# Autodesk Inventor assembly: Chassis-ver11-1111-2019
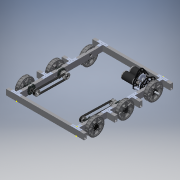
[picture p0: Inventor's stored thumbnail of the model, 180x180]
Saved by Autodesk Inventor 2018 (Build 220112000, 112)
## iProperties
Created: 2019-10-10
Part Number: Chassis-ver11-1111-2019
Document SubType Name: Assembly
Designer: JMHal
Author: JMHal
## Documents named in this file (26)
- E:\GrabCad\2020 Infinite Recharge\Chassis\Assembly\Chassis-ver11-1111-2019.iam
- E:\GrabCad\2020 Infinite Recharge\Chassis\Parts\2x1 20in Alluminum with Cal Drop.ver1-1111-2019.ipt
- E:\GrabCad\2020 Infinite Recharge\Chassis\Parts\2x1 20in Alluminum.ver1-1111-2019.ipt
- E:\GrabCad\2020 Infinite Recharge\Chassis\Parts\2x1 2in Alluminum Block.ver1-1111-2019.ipt
- E:\GrabCad\Resources\VEXpro Resources\Bearings\0.5inHexFlangedBearing(1.125inx0.313in)-1111-2016.ipt
- E:\GrabCad\Resources\VEXpro Resources\Versa Motion\VersaBlockKit-1111-2016.ipt
- E:\GrabCad\Resources\VEXpro Resources\Shafts\0.5inThunderHexShaft(8)-1111-2016.ipt
- E:\GrabCad\Resources\VEXpro Resources\Gearboxes\WCP SS Gearbox\SS-Gearbox.iam
- E:\GrabCad\Resources\VEXpro Resources\Gussets\ChassisGusset-1111-2016.ipt
- E:\GrabCad\2020 Infinite Recharge\Chassis\Parts\ElectricalBoard.ver1-1111-2019.ipt
- E:\GrabCad\Resources\VEXpro Resources\Spacers\0.5inAcetalSpace(0.5inHex)-1111-2016.ipt
- E:\GrabCad\Resources\VEXpro Resources\Spacers\0.5inAcetalSpace(0.5inHex)-1111-2016_MIR.ipt
- E:\GrabCad\Resources\VEXpro Resources\Versa Motion\Timing Pulleys\TimingPulley30T15mmDoubleFlange(0.5inHex)-1111-2017.ipt
- E:\GrabCad\Resources\VEXpro Resources\Spacers\0.25inAcetalSpacer(0.5inHex)-1111-2016.ipt
- E:\GrabCad\Resources\VEXpro Resources\Spacers\0.125inAcetalSpacer(0.5inHex)-1111-2016.ipt
- E:\GrabCad\Resources\VEXpro Resources\Spacers\0.0625inAcetalSpacer(0.5inHex)-1111-2016.ipt
- E:\GrabCad\Resources\VEXpro Resources\Spacers\1inAcetalSpacer(0.5inHex)-1111-2016.ipt
- E:\GrabCad\Resources\VEXpro Resources\Versa Motion\Timing Pulleys\TimingPulley30T15mmDoubleFlange(0.5inHex)-1111-2017_MIR.ipt
- E:\GrabCad\Resources\VEXpro Resources\Spacers\0.25inAcetalSpacer(0.5inHex)-1111-2016_MIR.ipt
- E:\GrabCad\Resources\VEXpro Resources\Spacers\0.125inAcetalSpacer(0.5inHex)-1111-2016_MIR.ipt
- E:\GrabCad\Resources\VEXpro Resources\Spacers\0.0625inAcetalSpacer(0.5inHex)-1111-2016_MIR.ipt
- E:\GrabCad\Resources\VEXpro Resources\Spacers\1inAcetalSpacer(0.5inHex)-1111-2016_MIR.ipt
- E:\GrabCad\2020 Infinite Recharge\Chassis\Parts\BeltVer1-1111-2019.ipt
- E:\GrabCad\Resources\VEXpro Resources\Wheels\6 inch\6x1inTractionWheel-1111-2016.iam
- E:\GrabCad\2020 Infinite Recharge\Chassis\Parts\Bumbers.ver1-1111-2019.ipt
- C:\Users\Demarcus\Desktop\WCDShiftingGearboxPTO.ver1-1111-2020.iam
## Components (69 placed, 25 different names)
1. 2x1 20in Alluminum with Cal Drop.ver1-1111-2019:1 — Mate:31, Mate:32, Insert:7, Mate:51, Insert:8, Angle:2, Mate:53, Angle:9, Insert:17, Angle:10, Insert:19, Angle:11, Mate:60, Cylindrical:1, Angle:16, Flush:1, Mate:65, Mate:66, Flush:2, Mate:67, Flush:4, Flush:5, Mate:77, Mate:78, Flush:16, Flush:17, Mate:80, Flush:20, Flush:23, Symmetry:1, Flush:43, Symmetry:2, Flush:62, Mate:141
2. 2x1 20in Alluminum.ver1-1111-2019:1 — Mate:65, Mate:66, Flush:2, Mate:68, Mate:72, Mate:81, Flush:22, Mate:82, Flush:24, Flush:44, Flush:62, Mate:140, Flush:63
3. 2x1 20in Alluminum with Cal Drop.ver1-1111-2019:2 — Insert:4, Insert:5, Angle:7, Angle:8, Insert:23, Angle:13, Insert:25, Angle:14, Flush:6, Flush:8, Mate:73, Flush:9, Flush:34, Flush:35, Flush:36, Flush:37, Symmetry:1, Symmetry:2, Cylindrical:42, Mate:142, Mate:143
4. 2x1 20in Alluminum.ver1-1111-2019:2 — Mate:67, Flush:4, Flush:5, Mate:69, Flush:6, Mate:71, Mate:73, Mate:79, Flush:19, Flush:21
5. 0.5inThunderHexShaft(8)-1111-2016:1 — Cylindrical:2, Cylindrical:18
6. SS-Gearbox:2 [sub-assembly] — Mate:60, Cylindrical:1, Angle:16
7. 0.5inThunderHexShaft(8)-1111-2016:2 — Cylindrical:3, Cylindrical:16, Flush:64
8. ChassisGusset-1111-2016:1 — Mate:76, Flush:12, Flush:36
9. ChassisGusset-1111-2016:2 — Mate:75, Flush:11, Flush:35
10. ChassisGusset-1111-2016:3 — Mate:78, Flush:14, Flush:17
11. ChassisGusset-1111-2016:4 — Mate:77, Flush:15, Flush:16
12. ChassisGusset-1111-2016:5 — Mate:82, Flush:24, Flush:34
13. ChassisGusset-1111-2016:6 — Mate:81, Flush:22, Flush:23
14. ChassisGusset-1111-2016:7 — Mate:80, Flush:20, Flush:21
15. ChassisGusset-1111-2016:8 — Mate:79, Flush:19, Flush:37
16. ElectricalBoard.ver1-1111-2019:1 — Flush:43, Flush:44
17. 0.5inAcetalSpace(0.5inHex)-1111-2016:1 — Cylindrical:16, Mate:89, Cylindrical:34, Mate:130
18. 0.5inAcetalSpace(0.5inHex)-1111-2016:2 — Cylindrical:18, Mate:91, Cylindrical:35, Mate:131
19. 0.25inAcetalSpacer(0.5inHex)-1111-2016:3 — Cylindrical:36, Mate:132
20. 0.5inAcetalSpace(0.5inHex)-1111-2016_MIR:1 — Mate:119, Rotational:14, Cylindrical:38, Mate:134
21. 0.5inAcetalSpace(0.5inHex)-1111-2016_MIR:2 — Cylindrical:31, Mate:127, Rotational:15
22. 0.25inAcetalSpacer(0.5inHex)-1111-2016:4 — Cylindrical:40, Mate:136
23. TimingPulley30T15mmDoubleFlange(0.5inHex)-1111-2017:1 — Rotational:7, Mate:117
24. TimingPulley30T15mmDoubleFlange(0.5inHex)-1111-2017:2 — Rotational:3
25. TimingPulley30T15mmDoubleFlange(0.5inHex)-1111-2017:3 — Cylindrical:25, Mate:111, Rotational:2
26. 0.25inAcetalSpacer(0.5inHex)-1111-2016:1 — Cylindrical:25, Cylindrical:26, Mate:109, Mate:110, Rotational:4
27. 0.125inAcetalSpacer(0.5inHex)-1111-2016:1 — Cylindrical:26, Mate:110, Mate:111
28. 0.0625inAcetalSpacer(0.5inHex)-1111-2016:1 — Rotational:2, Rotational:3
29. 0.25inAcetalSpacer(0.5inHex)-1111-2016:2 — Rotational:6, Rotational:7
30. 1inAcetalSpacer(0.5inHex)-1111-2016:1 — Rotational:5, Rotational:6
31. TimingPulley30T15mmDoubleFlange(0.5inHex)-1111-2017_MIR:1 — Rotational:10, Mate:114, Mate:115
32. TimingPulley30T15mmDoubleFlange(0.5inHex)-1111-2017_MIR:2 — Rotational:8, Cylindrical:30, Flush:60
33. TimingPulley30T15mmDoubleFlange(0.5inHex)-1111-2017_MIR:3 — Mate:112, Cylindrical:27, Rotational:9
34. 0.25inAcetalSpacer(0.5inHex)-1111-2016_MIR:1 — Mate:113, Cylindrical:27, Cylindrical:28, Rotational:12
35. 0.125inAcetalSpacer(0.5inHex)-1111-2016_MIR:1 — Mate:112, Mate:113, Cylindrical:28
36. 0.0625inAcetalSpacer(0.5inHex)-1111-2016_MIR:1 — Rotational:8, Rotational:9
37. 0.25inAcetalSpacer(0.5inHex)-1111-2016_MIR:2 — Rotational:10, Rotational:11
38. 1inAcetalSpacer(0.5inHex)-1111-2016_MIR:1 — Rotational:11, Rotational:13
39. BeltVer1-1111-2019:1 — Mate:114, Mate:115
40. BeltVer1-1111-2019:2 — Mate:117
41. 0.5inThunderHexShaft(8)-1111-2016:3 — Cylindrical:30, Flush:60, Cylindrical:31
42. 6x1inTractionWheel-1111-2016:1 [sub-assembly] — Cylindrical:34, Mate:130, Flush:64
43. 6x1inTractionWheel-1111-2016:2 [sub-assembly] — Cylindrical:35, Mate:131
44. 6x1inTractionWheel-1111-2016:3 [sub-assembly] — Cylindrical:36, Mate:132
45. 6x1inTractionWheel-1111-2016:5 [sub-assembly] — Cylindrical:38, Mate:134
46. 6x1inTractionWheel-1111-2016:6 [sub-assembly] — Cylindrical:40, Mate:136
47. 6x1inTractionWheel-1111-2016:8 [sub-assembly] — Rotational:15
48. Bumbers.ver1-1111-2019:1 — Mate:138, Mate:139, Mate:140
49. WCDShiftingGearboxPTO.ver1-1111-2020:1 [sub-assembly] — Cylindrical:42
50. 0.5inHexFlangedBearing(1.125inx0.313in)-1111-2016:20 — Rotational:12
51. 0.5inHexFlangedBearing(1.125inx0.313in)-1111-2016:19 — Rotational:13
52. 0.5inHexFlangedBearing(1.125inx0.313in)-1111-2016:6 — Insert:4, Mate:46, Mate:47, Mate:127
53. 0.5inHexFlangedBearing(1.125inx0.313in)-1111-2016:7 — Insert:5, Mate:48, Mate:49, Mate:119, Rotational:14
54. 0.5inHexFlangedBearing(1.125inx0.313in)-1111-2016:17 — Insert:19, Cylindrical:3, Rotational:5
55. 0.5inHexFlangedBearing(1.125inx0.313in)-1111-2016:16 — Insert:16, Insert:17, Cylindrical:2, Mate:109, Rotational:4
56. 0.5inHexFlangedBearing(1.125inx0.313in)-1111-2016:9 — Insert:7, Mate:50, Mate:91
57. 0.5inHexFlangedBearing(1.125inx0.313in)-1111-2016:10 — Insert:8, Mate:52, Mate:89
58. 2x1 2in Alluminum Block.ver1-1111-2019:5 — Mate:31, Mate:32, Mate:69, Flush:15
59. 2x1 2in Alluminum Block.ver1-1111-2019:6 — Flush:1, Mate:68, Flush:14, Mate:141
60. 2x1 2in Alluminum Block.ver1-1111-2019:7 — Mate:72, Flush:9, Mate:75, Flush:11, Mate:143, Flush:63
61. 2x1 2in Alluminum Block.ver1-1111-2019:8 — Flush:8, Mate:71, Mate:76, Flush:12, Mate:138, Mate:139, Mate:142
62. VersaBlockKit-1111-2016:2 — Mate:46, Mate:47, Angle:8
63. VersaBlockKit-1111-2016:3 — Mate:48, Mate:49, Angle:7
64. VersaBlockKit-1111-2016:5 — Mate:50, Mate:51, Angle:2
65. VersaBlockKit-1111-2016:6 — Mate:52, Mate:53, Angle:9
66. VersaBlockKit-1111-2016:8 — Insert:16, Angle:10
67. VersaBlockKit-1111-2016:9 — Angle:11
68. VersaBlockKit-1111-2016:11 — Insert:23, Angle:13
69. VersaBlockKit-1111-2016:12 — Insert:25, Angle:14
## Relationships (139: Mate 55, Flush 29, CylindricalJoint 18, RevoluteJoint 14, Insert 12, Angle 9, Symmetry 2)
- Mate:31: 2x1 20in Alluminum with Cal Drop.ver1-1111-2019:1 ↔ 2x1 2in Alluminum Block.ver1-1111-2019:5
- Mate:32: 2x1 20in Alluminum with Cal Drop.ver1-1111-2019:1 ↔ 2x1 2in Alluminum Block.ver1-1111-2019:5
- Insert:4: 2x1 20in Alluminum with Cal Drop.ver1-1111-2019:2 ↔ 0.5inHexFlangedBearing(1.125inx0.313in)-1111-2016:6
- Mate:46: 0.5inHexFlangedBearing(1.125inx0.313in)-1111-2016:6 ↔ VersaBlockKit-1111-2016:2
- Mate:47: 0.5inHexFlangedBearing(1.125inx0.313in)-1111-2016:6 ↔ VersaBlockKit-1111-2016:2
- Insert:5: 2x1 20in Alluminum with Cal Drop.ver1-1111-2019:2 ↔ 0.5inHexFlangedBearing(1.125inx0.313in)-1111-2016:7
- Mate:48: 0.5inHexFlangedBearing(1.125inx0.313in)-1111-2016:7 ↔ VersaBlockKit-1111-2016:3
- Mate:49: 0.5inHexFlangedBearing(1.125inx0.313in)-1111-2016:7 ↔ VersaBlockKit-1111-2016:3
- Insert:7: 2x1 20in Alluminum with Cal Drop.ver1-1111-2019:1 ↔ 0.5inHexFlangedBearing(1.125inx0.313in)-1111-2016:9
- Mate:50: 0.5inHexFlangedBearing(1.125inx0.313in)-1111-2016:9 ↔ VersaBlockKit-1111-2016:5
- Mate:51: 2x1 20in Alluminum with Cal Drop.ver1-1111-2019:1 ↔ VersaBlockKit-1111-2016:5
- Insert:8: 2x1 20in Alluminum with Cal Drop.ver1-1111-2019:1 ↔ 0.5inHexFlangedBearing(1.125inx0.313in)-1111-2016:10
- Angle:2 (0 deg): 2x1 20in Alluminum with Cal Drop.ver1-1111-2019:1 ↔ VersaBlockKit-1111-2016:5
- Angle:7 (0 deg): 2x1 20in Alluminum with Cal Drop.ver1-1111-2019:2 ↔ VersaBlockKit-1111-2016:3
- Angle:8 (0 deg): 2x1 20in Alluminum with Cal Drop.ver1-1111-2019:2 ↔ VersaBlockKit-1111-2016:2
- Mate:52: 0.5inHexFlangedBearing(1.125inx0.313in)-1111-2016:10 ↔ VersaBlockKit-1111-2016:6
- Mate:53: 2x1 20in Alluminum with Cal Drop.ver1-1111-2019:1 ↔ VersaBlockKit-1111-2016:6
- Angle:9 (0 deg): 2x1 20in Alluminum with Cal Drop.ver1-1111-2019:1 ↔ VersaBlockKit-1111-2016:6
- [Mate]: 0.5inHexFlangedBearing(1.125inx0.313in)-1111-2016:16 ↔ VersaBlockKit-1111-2016:8
- Insert:16: 0.5inHexFlangedBearing(1.125inx0.313in)-1111-2016:16 ↔ VersaBlockKit-1111-2016:8
- Insert:17: 2x1 20in Alluminum with Cal Drop.ver1-1111-2019:1 ↔ 0.5inHexFlangedBearing(1.125inx0.313in)-1111-2016:16
- Angle:10 (0 deg): 2x1 20in Alluminum with Cal Drop.ver1-1111-2019:1 ↔ VersaBlockKit-1111-2016:8
- [Mate]: 0.5inHexFlangedBearing(1.125inx0.313in)-1111-2016:17 ↔ VersaBlockKit-1111-2016:9
- [Insert]: 0.5inHexFlangedBearing(1.125inx0.313in)-1111-2016:17 ↔ VersaBlockKit-1111-2016:9
- Insert:19: 2x1 20in Alluminum with Cal Drop.ver1-1111-2019:1 ↔ 0.5inHexFlangedBearing(1.125inx0.313in)-1111-2016:17
- Angle:11 (0 deg): 2x1 20in Alluminum with Cal Drop.ver1-1111-2019:1 ↔ VersaBlockKit-1111-2016:9
- [Mate]: 0.5inHexFlangedBearing(1.125inx0.313in)-1111-2016:19 ↔ VersaBlockKit-1111-2016:11
- [Insert]: 0.5inHexFlangedBearing(1.125inx0.313in)-1111-2016:19 ↔ VersaBlockKit-1111-2016:11
- Insert:23: 2x1 20in Alluminum with Cal Drop.ver1-1111-2019:2 ↔ VersaBlockKit-1111-2016:11
- Angle:13 (0 deg): 2x1 20in Alluminum with Cal Drop.ver1-1111-2019:2 ↔ VersaBlockKit-1111-2016:11
- [Mate]: 0.5inHexFlangedBearing(1.125inx0.313in)-1111-2016:20 ↔ VersaBlockKit-1111-2016:12
- [Insert]: 0.5inHexFlangedBearing(1.125inx0.313in)-1111-2016:20 ↔ VersaBlockKit-1111-2016:12
- Insert:25: 2x1 20in Alluminum with Cal Drop.ver1-1111-2019:2 ↔ VersaBlockKit-1111-2016:12
- Angle:14 (0 deg): 2x1 20in Alluminum with Cal Drop.ver1-1111-2019:2 ↔ VersaBlockKit-1111-2016:12
- Mate:60: 2x1 20in Alluminum with Cal Drop.ver1-1111-2019:1 ↔ SS-Gearbox:2
- Cylindrical:1: 2x1 20in Alluminum with Cal Drop.ver1-1111-2019:1 ↔ SS-Gearbox:2
- Cylindrical:2: 0.5inThunderHexShaft(8)-1111-2016:1 ↔ 0.5inHexFlangedBearing(1.125inx0.313in)-1111-2016:16
- Cylindrical:3: 0.5inThunderHexShaft(8)-1111-2016:2 ↔ 0.5inHexFlangedBearing(1.125inx0.313in)-1111-2016:17
- Angle:16 (90 deg): 2x1 20in Alluminum with Cal Drop.ver1-1111-2019:1 ↔ SS-Gearbox:2
- Flush:1: 2x1 20in Alluminum with Cal Drop.ver1-1111-2019:1 ↔ 2x1 2in Alluminum Block.ver1-1111-2019:6
- Mate:65: 2x1 20in Alluminum with Cal Drop.ver1-1111-2019:1 ↔ 2x1 20in Alluminum.ver1-1111-2019:1
- Mate:66: 2x1 20in Alluminum with Cal Drop.ver1-1111-2019:1 ↔ 2x1 20in Alluminum.ver1-1111-2019:1
- Flush:2: 2x1 20in Alluminum with Cal Drop.ver1-1111-2019:1 ↔ 2x1 20in Alluminum.ver1-1111-2019:1
- Mate:67: 2x1 20in Alluminum with Cal Drop.ver1-1111-2019:1 ↔ 2x1 20in Alluminum.ver1-1111-2019:2
- Flush:4: 2x1 20in Alluminum with Cal Drop.ver1-1111-2019:1 ↔ 2x1 20in Alluminum.ver1-1111-2019:2
- Flush:5 (-69.85 mm): 2x1 20in Alluminum with Cal Drop.ver1-1111-2019:1 ↔ 2x1 20in Alluminum.ver1-1111-2019:2
- Mate:68 (254 mm): 2x1 20in Alluminum.ver1-1111-2019:1 ↔ 2x1 2in Alluminum Block.ver1-1111-2019:6
- Mate:69 (254 mm): 2x1 20in Alluminum.ver1-1111-2019:2 ↔ 2x1 2in Alluminum Block.ver1-1111-2019:5
- Flush:6: 2x1 20in Alluminum with Cal Drop.ver1-1111-2019:2 ↔ 2x1 20in Alluminum.ver1-1111-2019:2
- Flush:8: 2x1 20in Alluminum with Cal Drop.ver1-1111-2019:2 ↔ 2x1 2in Alluminum Block.ver1-1111-2019:8
- Mate:71 (254 mm): 2x1 20in Alluminum.ver1-1111-2019:2 ↔ 2x1 2in Alluminum Block.ver1-1111-2019:8
- Mate:72 (254 mm): 2x1 20in Alluminum.ver1-1111-2019:1 ↔ 2x1 2in Alluminum Block.ver1-1111-2019:7
- Mate:73: 2x1 20in Alluminum with Cal Drop.ver1-1111-2019:2 ↔ 2x1 20in Alluminum.ver1-1111-2019:2
- Flush:9: 2x1 20in Alluminum with Cal Drop.ver1-1111-2019:2 ↔ 2x1 2in Alluminum Block.ver1-1111-2019:7
- Mate:75: ChassisGusset-1111-2016:2 ↔ 2x1 2in Alluminum Block.ver1-1111-2019:7
- Flush:11: ChassisGusset-1111-2016:2 ↔ 2x1 2in Alluminum Block.ver1-1111-2019:7
- Mate:76: ChassisGusset-1111-2016:1 ↔ 2x1 2in Alluminum Block.ver1-1111-2019:8
- Flush:12: ChassisGusset-1111-2016:1 ↔ 2x1 2in Alluminum Block.ver1-1111-2019:8
- Mate:77: 2x1 20in Alluminum with Cal Drop.ver1-1111-2019:1 ↔ ChassisGusset-1111-2016:4
- Mate:78: 2x1 20in Alluminum with Cal Drop.ver1-1111-2019:1 ↔ ChassisGusset-1111-2016:3
- Flush:14: ChassisGusset-1111-2016:3 ↔ 2x1 2in Alluminum Block.ver1-1111-2019:6
- Flush:15: ChassisGusset-1111-2016:4 ↔ 2x1 2in Alluminum Block.ver1-1111-2019:5
- Flush:16: 2x1 20in Alluminum with Cal Drop.ver1-1111-2019:1 ↔ ChassisGusset-1111-2016:4
- Flush:17: 2x1 20in Alluminum with Cal Drop.ver1-1111-2019:1 ↔ ChassisGusset-1111-2016:3
- Mate:79: 2x1 20in Alluminum.ver1-1111-2019:2 ↔ ChassisGusset-1111-2016:8
- Flush:19: 2x1 20in Alluminum.ver1-1111-2019:2 ↔ ChassisGusset-1111-2016:8
- Mate:80: 2x1 20in Alluminum with Cal Drop.ver1-1111-2019:1 ↔ ChassisGusset-1111-2016:7
- Flush:20: 2x1 20in Alluminum with Cal Drop.ver1-1111-2019:1 ↔ ChassisGusset-1111-2016:7
- Flush:21: 2x1 20in Alluminum.ver1-1111-2019:2 ↔ ChassisGusset-1111-2016:7
- Mate:81: 2x1 20in Alluminum.ver1-1111-2019:1 ↔ ChassisGusset-1111-2016:6
- Flush:22: 2x1 20in Alluminum.ver1-1111-2019:1 ↔ ChassisGusset-1111-2016:6
- Flush:23: 2x1 20in Alluminum with Cal Drop.ver1-1111-2019:1 ↔ ChassisGusset-1111-2016:6
- Mate:82: 2x1 20in Alluminum.ver1-1111-2019:1 ↔ ChassisGusset-1111-2016:5
- Flush:24: 2x1 20in Alluminum.ver1-1111-2019:1 ↔ ChassisGusset-1111-2016:5
- Flush:34: 2x1 20in Alluminum with Cal Drop.ver1-1111-2019:2 ↔ ChassisGusset-1111-2016:5
- Flush:35: 2x1 20in Alluminum with Cal Drop.ver1-1111-2019:2 ↔ ChassisGusset-1111-2016:2
- Flush:36: 2x1 20in Alluminum with Cal Drop.ver1-1111-2019:2 ↔ ChassisGusset-1111-2016:1
- Flush:37: 2x1 20in Alluminum with Cal Drop.ver1-1111-2019:2 ↔ ChassisGusset-1111-2016:8
- Cylindrical:16: 0.5inThunderHexShaft(8)-1111-2016:2 ↔ 0.5inAcetalSpace(0.5inHex)-1111-2016:1
- Mate:89: 0.5inAcetalSpace(0.5inHex)-1111-2016:1 ↔ 0.5inHexFlangedBearing(1.125inx0.313in)-1111-2016:10
- Cylindrical:18: 0.5inThunderHexShaft(8)-1111-2016:1 ↔ 0.5inAcetalSpace(0.5inHex)-1111-2016:2
- Mate:91: 0.5inAcetalSpace(0.5inHex)-1111-2016:2 ↔ 0.5inHexFlangedBearing(1.125inx0.313in)-1111-2016:9
- [CylindricalJoint]: SS-Gearbox:2 ↔ 0.25inAcetalSpacer(0.5inHex)-1111-2016:3
- [Mate]: SS-Gearbox:2 ↔ 0.25inAcetalSpacer(0.5inHex)-1111-2016:3
- Symmetry:1: 2x1 20in Alluminum with Cal Drop.ver1-1111-2019:1 ↔ 2x1 20in Alluminum with Cal Drop.ver1-1111-2019:2
- Flush:43: 2x1 20in Alluminum with Cal Drop.ver1-1111-2019:1 ↔ ElectricalBoard.ver1-1111-2019:1
- Flush:44: 2x1 20in Alluminum.ver1-1111-2019:1 ↔ ElectricalBoard.ver1-1111-2019:1
- Cylindrical:25: TimingPulley30T15mmDoubleFlange(0.5inHex)-1111-2017:3 ↔ 0.25inAcetalSpacer(0.5inHex)-1111-2016:1
- Cylindrical:26: 0.25inAcetalSpacer(0.5inHex)-1111-2016:1 ↔ 0.125inAcetalSpacer(0.5inHex)-1111-2016:1
- Mate:109: 0.25inAcetalSpacer(0.5inHex)-1111-2016:1 ↔ 0.5inHexFlangedBearing(1.125inx0.313in)-1111-2016:16
- Mate:110: 0.25inAcetalSpacer(0.5inHex)-1111-2016:1 ↔ 0.125inAcetalSpacer(0.5inHex)-1111-2016:1
- Mate:111: TimingPulley30T15mmDoubleFlange(0.5inHex)-1111-2017:3 ↔ 0.125inAcetalSpacer(0.5inHex)-1111-2016:1
- Rotational:2 [RevoluteJoint]: TimingPulley30T15mmDoubleFlange(0.5inHex)-1111-2017:3 ↔ 0.0625inAcetalSpacer(0.5inHex)-1111-2016:1
- Rotational:3 [RevoluteJoint]: TimingPulley30T15mmDoubleFlange(0.5inHex)-1111-2017:2 ↔ 0.0625inAcetalSpacer(0.5inHex)-1111-2016:1
- Rotational:4 [RevoluteJoint]: 0.25inAcetalSpacer(0.5inHex)-1111-2016:1 ↔ 0.5inHexFlangedBearing(1.125inx0.313in)-1111-2016:16
- Rotational:5 [RevoluteJoint]: 1inAcetalSpacer(0.5inHex)-1111-2016:1 ↔ 0.5inHexFlangedBearing(1.125inx0.313in)-1111-2016:17
- Rotational:6 [RevoluteJoint]: 0.25inAcetalSpacer(0.5inHex)-1111-2016:2 ↔ 1inAcetalSpacer(0.5inHex)-1111-2016:1
- Rotational:7 [RevoluteJoint]: TimingPulley30T15mmDoubleFlange(0.5inHex)-1111-2017:1 ↔ 0.25inAcetalSpacer(0.5inHex)-1111-2016:2
- Symmetry:2: 2x1 20in Alluminum with Cal Drop.ver1-1111-2019:1 ↔ 2x1 20in Alluminum with Cal Drop.ver1-1111-2019:2
- Mate:112: TimingPulley30T15mmDoubleFlange(0.5inHex)-1111-2017_MIR:3 ↔ 0.125inAcetalSpacer(0.5inHex)-1111-2016_MIR:1
- Mate:113: 0.25inAcetalSpacer(0.5inHex)-1111-2016_MIR:1 ↔ 0.125inAcetalSpacer(0.5inHex)-1111-2016_MIR:1
- Cylindrical:27: TimingPulley30T15mmDoubleFlange(0.5inHex)-1111-2017_MIR:3 ↔ 0.25inAcetalSpacer(0.5inHex)-1111-2016_MIR:1
- Cylindrical:28: 0.25inAcetalSpacer(0.5inHex)-1111-2016_MIR:1 ↔ 0.125inAcetalSpacer(0.5inHex)-1111-2016_MIR:1
- Rotational:8 [RevoluteJoint]: TimingPulley30T15mmDoubleFlange(0.5inHex)-1111-2017_MIR:2 ↔ 0.0625inAcetalSpacer(0.5inHex)-1111-2016_MIR:1
- Rotational:9 [RevoluteJoint]: TimingPulley30T15mmDoubleFlange(0.5inHex)-1111-2017_MIR:3 ↔ 0.0625inAcetalSpacer(0.5inHex)-1111-2016_MIR:1
- Rotational:10 [RevoluteJoint]: TimingPulley30T15mmDoubleFlange(0.5inHex)-1111-2017_MIR:1 ↔ 0.25inAcetalSpacer(0.5inHex)-1111-2016_MIR:2
- Rotational:11 [RevoluteJoint]: 0.25inAcetalSpacer(0.5inHex)-1111-2016_MIR:2 ↔ 1inAcetalSpacer(0.5inHex)-1111-2016_MIR:1
- Rotational:12 [RevoluteJoint]: 0.25inAcetalSpacer(0.5inHex)-1111-2016_MIR:1 ↔ 0.5inHexFlangedBearing(1.125inx0.313in)-1111-2016:20
- Rotational:13 [RevoluteJoint]: 1inAcetalSpacer(0.5inHex)-1111-2016_MIR:1 ↔ 0.5inHexFlangedBearing(1.125inx0.313in)-1111-2016:19
- Mate:114: TimingPulley30T15mmDoubleFlange(0.5inHex)-1111-2017_MIR:1 ↔ BeltVer1-1111-2019:1
- Mate:115: TimingPulley30T15mmDoubleFlange(0.5inHex)-1111-2017_MIR:1 ↔ BeltVer1-1111-2019:1
- Mate:117: TimingPulley30T15mmDoubleFlange(0.5inHex)-1111-2017:1 ↔ BeltVer1-1111-2019:2
- Mate:119: 0.5inAcetalSpace(0.5inHex)-1111-2016_MIR:1 ↔ 0.5inHexFlangedBearing(1.125inx0.313in)-1111-2016:7
- Rotational:14 [RevoluteJoint]: 0.5inAcetalSpace(0.5inHex)-1111-2016_MIR:1 ↔ 0.5inHexFlangedBearing(1.125inx0.313in)-1111-2016:7
- Cylindrical:30: TimingPulley30T15mmDoubleFlange(0.5inHex)-1111-2017_MIR:2 ↔ 0.5inThunderHexShaft(8)-1111-2016:3
- Flush:60: TimingPulley30T15mmDoubleFlange(0.5inHex)-1111-2017_MIR:2 ↔ 0.5inThunderHexShaft(8)-1111-2016:3
- Flush:62 (69.85 mm): 2x1 20in Alluminum with Cal Drop.ver1-1111-2019:1 ↔ 2x1 20in Alluminum.ver1-1111-2019:1
- Cylindrical:31: 0.5inAcetalSpace(0.5inHex)-1111-2016_MIR:2 ↔ 0.5inThunderHexShaft(8)-1111-2016:3
- Mate:127: 0.5inAcetalSpace(0.5inHex)-1111-2016_MIR:2 ↔ 0.5inHexFlangedBearing(1.125inx0.313in)-1111-2016:6
- Cylindrical:34: 0.5inAcetalSpace(0.5inHex)-1111-2016:1 ↔ 6x1inTractionWheel-1111-2016:1
- Mate:130: 0.5inAcetalSpace(0.5inHex)-1111-2016:1 ↔ 6x1inTractionWheel-1111-2016:1
- Cylindrical:35: 0.5inAcetalSpace(0.5inHex)-1111-2016:2 ↔ 6x1inTractionWheel-1111-2016:2
- Mate:131: 0.5inAcetalSpace(0.5inHex)-1111-2016:2 ↔ 6x1inTractionWheel-1111-2016:2
- Cylindrical:36: 0.25inAcetalSpacer(0.5inHex)-1111-2016:3 ↔ 6x1inTractionWheel-1111-2016:3
- Mate:132: 0.25inAcetalSpacer(0.5inHex)-1111-2016:3 ↔ 6x1inTractionWheel-1111-2016:3
- Cylindrical:38: 0.5inAcetalSpace(0.5inHex)-1111-2016_MIR:1 ↔ 6x1inTractionWheel-1111-2016:5
- Mate:134: 0.5inAcetalSpace(0.5inHex)-1111-2016_MIR:1 ↔ 6x1inTractionWheel-1111-2016:5
- Rotational:15 [RevoluteJoint]: 0.5inAcetalSpace(0.5inHex)-1111-2016_MIR:2 ↔ 6x1inTractionWheel-1111-2016:8
- Cylindrical:40: 0.25inAcetalSpacer(0.5inHex)-1111-2016:4 ↔ 6x1inTractionWheel-1111-2016:6
- Mate:136: 0.25inAcetalSpacer(0.5inHex)-1111-2016:4 ↔ 6x1inTractionWheel-1111-2016:6
- Mate:138: Bumbers.ver1-1111-2019:1 ↔ 2x1 2in Alluminum Block.ver1-1111-2019:8
- Mate:139 (-127 mm): Bumbers.ver1-1111-2019:1 ↔ 2x1 2in Alluminum Block.ver1-1111-2019:8
- Mate:140: 2x1 20in Alluminum.ver1-1111-2019:1 ↔ Bumbers.ver1-1111-2019:1
- Cylindrical:42: 2x1 20in Alluminum with Cal Drop.ver1-1111-2019:2 ↔ WCDShiftingGearboxPTO.ver1-1111-2020:1
- Mate:141: 2x1 20in Alluminum with Cal Drop.ver1-1111-2019:1 ↔ 2x1 2in Alluminum Block.ver1-1111-2019:6
- Mate:142: 2x1 20in Alluminum with Cal Drop.ver1-1111-2019:2 ↔ 2x1 2in Alluminum Block.ver1-1111-2019:8
- Mate:143: 2x1 20in Alluminum with Cal Drop.ver1-1111-2019:2 ↔ 2x1 2in Alluminum Block.ver1-1111-2019:7
- Flush:63: 2x1 20in Alluminum.ver1-1111-2019:1 ↔ 2x1 2in Alluminum Block.ver1-1111-2019:7
- Flush:64: 0.5inThunderHexShaft(8)-1111-2016:2 ↔ 6x1inTractionWheel-1111-2016:1
## Named parameters: d89_d76 = 0 mm, d93_d89_d76 = 0 mm, d94_d90 = 0 mm, d103_d89_d76 = 0 mm, d104_d90 = 0 mm, d107_d89_d76 = 0 mm, d108_d90 = 0 mm
